# Autodesk Inventor assembly: Base
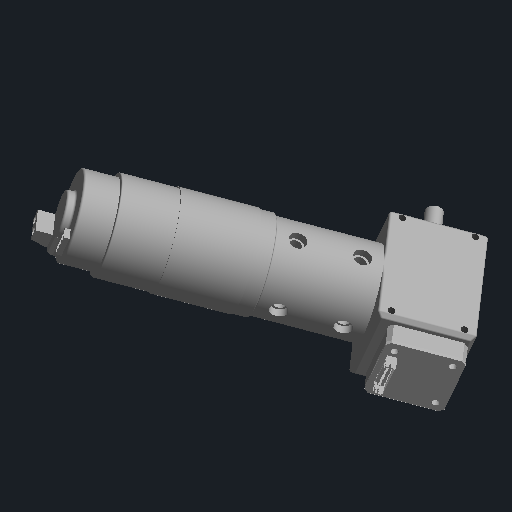
[picture p0: Inventor's stored thumbnail of the model, 512x512]
Saved by Autodesk Inventor 2025.2 (Build 292293000, 293)
## iProperties
Created: 2020-03-24
Part Number: Base
Document SubType Name: Assembly
Designer: valer
Mass: 715.256 g
Surface Area: 821.775 cm^2
Volume: 200.817 cm^3
Density: 3.56173 g/cm^3
Author: valer
## Documents named in this file (7)
- C:\Users\valer\Desktop\str1ker\cad\ArmBase.iam
- C:\Users\valer\Desktop\str1ker\cad\external\ShoulderActuator\DumaDynamics00E.ipt
- C:\Users\valer\Desktop\str1ker\cad\ShoulderEncoderSpacer.ipt
- C:\Users\valer\Desktop\str1ker\cad\external\ShoulderEncoder\ArmEncoderBoard.ipt
- C:\Users\valer\Desktop\str1ker\cad\external\ArmEncoder\ArmEncoderShaftMagnet6mm.ipt
- C:\Users\valer\Desktop\str1ker\cad\ShoulderEncoderFlange.ipt
- C:\Users\valer\Desktop\str1ker\cad\BaseBoundingBox.ipt
## Components (6 placed, 6 different names)
1. DumaDynamics00E:1 — Flush:1, Mate:16, Mate:17, Mate:36, Mate:37, Mate:38, Flush:5, Mate:39
2. ShoulderEncoderSpacer:1 — Mate:27, Mate:28, Mate:29, Mate:38
3. ArmEncoderBoard:1 — Mate:27, Mate:28, Mate:29, Mate:36, Mate:37
4. ArmEncoderShaftMagnet6mm:1 — Mate:16, Mate:17, Mate:25, Flush:4
5. ShoulderEncoderFlange:1 — Mate:25, Flush:4
6. BaseBoundingBox:1 — Mate:40
## Relationships (14: Mate 11, Flush 3)
- Flush:1: DumaDynamics00E:1
- Mate:16: DumaDynamics00E:1 ↔ ArmEncoderShaftMagnet6mm:1
- Mate:17: DumaDynamics00E:1 ↔ ArmEncoderShaftMagnet6mm:1
- Mate:25: ArmEncoderShaftMagnet6mm:1 ↔ ShoulderEncoderFlange:1
- Flush:4: ArmEncoderShaftMagnet6mm:1 ↔ ShoulderEncoderFlange:1
- Mate:27: ShoulderEncoderSpacer:1 ↔ ArmEncoderBoard:1
- Mate:28: ShoulderEncoderSpacer:1 ↔ ArmEncoderBoard:1
- Mate:29: ShoulderEncoderSpacer:1 ↔ ArmEncoderBoard:1
- Mate:36: DumaDynamics00E:1 ↔ ArmEncoderBoard:1
- Mate:37: DumaDynamics00E:1 ↔ ArmEncoderBoard:1
- Mate:38: DumaDynamics00E:1 ↔ ShoulderEncoderSpacer:1
- Flush:5 (6 mm): DumaDynamics00E:1
- Mate:39: DumaDynamics00E:1
- Mate:40: BaseBoundingBox:1
